# Autodesk Inventor assembly: #Spindexer
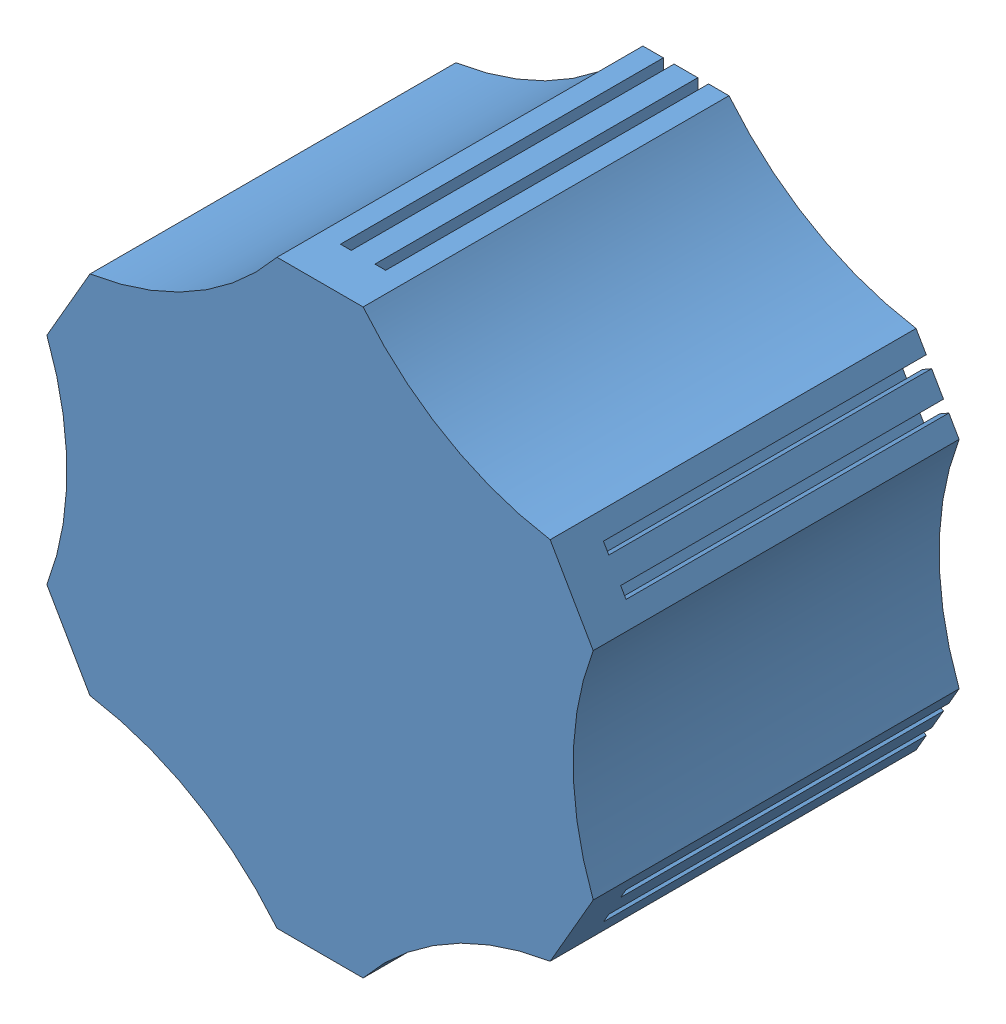
[picture p0: shaded view drawn from the shape stored in the file]
Saved by Autodesk Inventor 2026.1 (Build 301233020, 233B)
## iProperties
Created: 2026-02-05
Part Number: #Spindexer
Document SubType Name: Assembly
Designer: Owen L
Author: Owen L
## Documents named in this file (3)
- C:\Users\Owen\Documents\GitHub\2026-Robot-Mechanical\Spindexer\#Spindexer.iam
- C:\Users\Owen\Documents\GitHub\2026-Robot-Mechanical\Spindexer\TEMP,BASE-SKETCH.ipt
- C:\Users\Owen\Documents\GitHub\2026-Robot-Mechanical\Spindexer\3DPRINT,HUB.ipt
## Components (2 placed, 2 different names)
1. TEMP,BASE-SKETCH:1
2. 3DPRINT,HUB:1 — Mate:4
## Relationships (1: Mate 1)
- Mate:4: 3DPRINT,HUB:1
